# Autodesk Inventor assembly: fight_robot
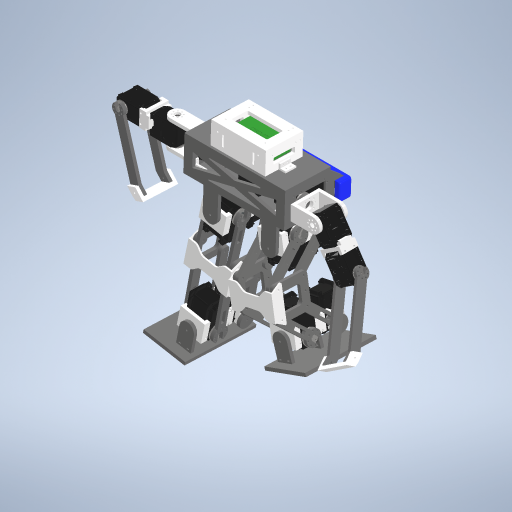
[picture p0: Inventor's stored thumbnail of the model, 512x512]
Saved by Autodesk Inventor 2024.3 (Build 283343000, 343)
## iProperties
Created: 2024-09-18
Part Number: fight_robot
Document SubType Name: Assembly
Designer: 구지현
Author: 구지현
## Documents named in this file (7)
- C:\Users\구지현\Desktop\19th_intern_kdy_fight_robot\부품\fight_robot.iam
- C:\Users\구지현\Desktop\19th_intern_kdy_fight_robot\부품\Upper_Body\Body\body.iam
- C:\Users\구지현\Desktop\19th_intern_kdy_fight_robot\부품\Upper_Body\Arm\Arm_Left.iam
- C:\Users\구지현\Desktop\19th_intern_kdy_fight_robot\부품\Upper_Body\Arm\Arm_Right.iam
- C:\Users\구지현\Desktop\19th_intern_kdy_fight_robot\부품\Lower_Body\Hip\Hip.iam
- C:\Users\구지현\Desktop\19th_intern_kdy_fight_robot\부품\Lower_Body\Leg\Leg_left.iam
- C:\Users\구지현\Desktop\19th_intern_kdy_fight_robot\부품\Lower_Body\Leg\Leg_Right.iam
## Components (6 placed, 6 different names)
1. body:1 [sub-assembly] — 삽입:1, 삽입:2, 삽입:3, 삽입:4, 삽입:6
2. Arm_Left:1 [sub-assembly] — 삽입:1, 삽입:2
3. Arm_Right:1 [sub-assembly] — 삽입:3, 삽입:4
4. Hip:1 [sub-assembly] — 삽입:5, 삽입:6, 삽입:7
5. Leg_left:1 [sub-assembly] — 삽입:5
6. Leg_Right:1 [sub-assembly] — 삽입:7
## Relationships (7: Insert 7)
- 삽입:1 [Insert]: body:1 ↔ Arm_Left:1
- 삽입:2 [Insert]: body:1 ↔ Arm_Left:1
- 삽입:3 [Insert]: body:1 ↔ Arm_Right:1
- 삽입:4 [Insert]: body:1 ↔ Arm_Right:1
- 삽입:5 [Insert]: Hip:1 ↔ Leg_left:1
- 삽입:6 [Insert]: body:1 ↔ Hip:1
- 삽입:7 [Insert]: Hip:1 ↔ Leg_Right:1
